# Autodesk Inventor assembly: Final_Skeleton
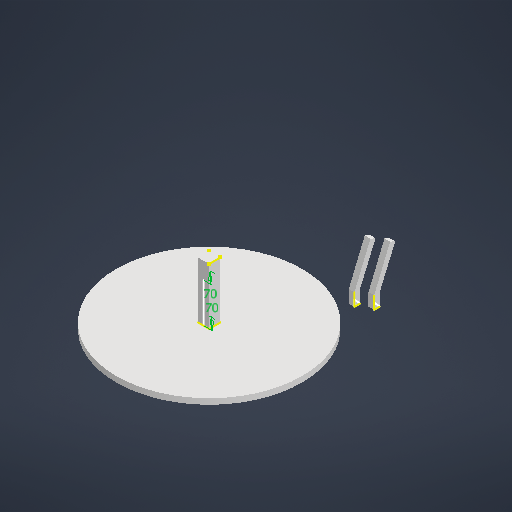
[picture p0: Inventor's stored thumbnail of the model, 512x512]
Saved by Autodesk Inventor 2026.1 (Build 301233000, 233)
## iProperties
Created: 2025-09-01
Part Number: Final_Skeleton
Document SubType Name: Assembly
Designer: junha
Author: junha
## Documents named in this file (4)
- C:\Users\junha\Downloads\Skeleton\Final_Skeleton.iam
- C:\Users\junha\Downloads\Skeleton\Main_Base.ipt
- C:\Users\junha\Downloads\Skeleton\Main_Pole.ipt
- C:\Users\junha\Downloads\Skeleton\Arm_Servo_Cone.ipt
## Components (4 placed, 3 different names)
1. Main_Base:1 — Rigid:1
2. Arm_Servo_Cone:1
3. Arm_Servo_Cone:2
4. Main_Pole:1 — Rigid:1
## Relationships (1: WeldJoint 1)
- Rigid:1 [WeldJoint]: Main_Base:1 ↔ Main_Pole:1
